# Autodesk Inventor assembly: złożenie czołg
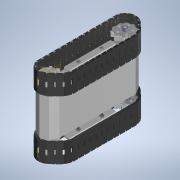
[picture p0: Inventor's stored thumbnail of the model, 180x180]
Saved by Autodesk Inventor 2021 (Build 250183000, 183)
## iProperties
Created: 2021-06-22
Part Number: złożenie czołg
Document SubType Name: Assembly
Designer: Łukasz
Author: Łukasz
## Documents named in this file (10)
- E:\GITHUB_Czołg\Szybki-Czolg-antyRadziecki\złożenie czołg.iam
- E:\GITHUB_Czołg\Szybki-Czolg-antyRadziecki\złożenie gąsienicy lewej.iam
- E:\GITHUB_Czołg\Szybki-Czolg-antyRadziecki\złożenie gąsienicy prawej.iam
- C:\Users\Łukasz\Documents\Inventor\Content Center Files\R2021\en-US\AS 1237 (3.1)\AS 1237 - 12 mm(1)Aluminium-6061.ipt
- C:\Users\Łukasz\Documents\Inventor\Content Center Files\R2021\en-US\BS 292 (I)\BS 292 Part 1 - 6001 - 12 x 28 x 8.ipt
- E:\GITHUB_Czołg\Szybki-Czolg-antyRadziecki\rama.ipt
- E:\GITHUB_Czołg\Szybki-Czolg-antyRadziecki\dystans na łożysk 6001 19mm.ipt
- E:\GITHUB_Czołg\Szybki-Czolg-antyRadziecki\blokada osi.ipt
- C:\Users\Łukasz\Documents\Inventor\Content Center Files\R2021\en-US\KS B 1002  C (2)\KS B 1002 - C  M 8 x 60(1).ipt
- C:\Users\Łukasz\Documents\Inventor\Content Center Files\R2021\en-US\AS 1474(1)\AS 1474 - M8(1).ipt
## Components (31 placed, 9 different names)
1. złożenie gąsienicy lewej:1 [sub-assembly] — Flush:2, Flush:3, Mate:1, Rotational:1, Rotational:10, Rotational:11, Rotational:17, Rotational:18, Rotational:19, Rotational:20
2. złożenie gąsienicy prawej:1 [sub-assembly] — Flush:2, Flush:3, Mate:1, Rigid:1, Angle:1, Rotational:6, Rotational:7, Rotational:21, Rotational:22, Rotational:25, Rotational:26
3. AS 1237 (3.1) 12 mm - Aluminum 6061:1 — Rigid:1, Rotational:5
4. AS 1237 (3.1) 12 mm - Aluminum 6061:2 — Rotational:1
5. BS 292: Part 1 (I) (Metric) 6001 - 12 x 28 x 8:1 — Rotational:2, Rotational:3, Rotational:5
6. BS 292: Part 1 (I) (Metric) 6001 - 12 x 28 x 8:2 — Rotational:4
7. rama:1 — Rotational:2, Angle:1, Rigid:2, Rigid:3, Rotational:12, Rotational:13, Rotational:14, Rotational:15, Rotational:16, Rotational:23, Rotational:24
8. dystans na łożysk 6001 19mm:1 — Rotational:3, Rotational:4
9. blokada osi:1 — Rotational:6
10. blokada osi:2 — Rotational:7
11. dystans na łożysk 6001 19mm:2 — Rotational:8, Rotational:9
12. BS 292: Part 1 (I) (Metric) 6001 - 12 x 28 x 8:3 — Rotational:9
13. BS 292: Part 1 (I) (Metric) 6001 - 12 x 28 x 8:4 — Rigid:2, Rotational:8
14. blokada osi:3 — Rotational:11
15. blokada osi:4 — Rotational:10
16. KS B 1002 C Regular Thread (Full Threaded) C  M 8 x 60:1 — Rotational:12
17. KS B 1002 C Regular Thread (Full Threaded) C  M 8 x 60:2 — Rotational:14
18. KS B 1002 C Regular Thread (Full Threaded) C  M 8 x 60:3 — Rigid:3
19. KS B 1002 C Regular Thread (Full Threaded) C  M 8 x 60:4 — Rotational:13
20. AS 1474 - Metric M8:1 — Rotational:20
21. AS 1474 - Metric M8:2 — Rotational:21
22. AS 1474 - Metric M8:3 — Rotational:23
23. AS 1474 - Metric M8:4 — Rotational:22
24. AS 1474 - Metric M8:5 — Rotational:26
25. AS 1474 - Metric M8:6 — Rotational:24
26. AS 1474 - Metric M8:7 — Rotational:19
27. AS 1474 - Metric M8:8 — Rotational:25
28. AS 1474 - Metric M8:9 — Rotational:17
29. AS 1474 - Metric M8:10 — Rotational:18
30. AS 1474 - Metric M8:11 — Rotational:15
31. AS 1474 - Metric M8:12 — Rotational:16
## Relationships (33: RevoluteJoint 26, WeldJoint 3, Flush 2, Mate 1, Angle 1)
- Flush:2: złożenie gąsienicy lewej:1 ↔ złożenie gąsienicy prawej:1
- Flush:3: złożenie gąsienicy lewej:1 ↔ złożenie gąsienicy prawej:1
- Mate:1 (170 mm): złożenie gąsienicy lewej:1 ↔ złożenie gąsienicy prawej:1
- Rigid:1 [WeldJoint]: złożenie gąsienicy prawej:1 ↔ AS 1237 (3.1) 12 mm - Aluminum 6061:1
- Rotational:1 [RevoluteJoint]: złożenie gąsienicy lewej:1 ↔ AS 1237 (3.1) 12 mm - Aluminum 6061:2
- Rotational:2 [RevoluteJoint]: BS 292: Part 1 (I) (Metric) 6001 - 12 x 28 x 8:1 ↔ rama:1
- Rotational:3 [RevoluteJoint]: BS 292: Part 1 (I) (Metric) 6001 - 12 x 28 x 8:1 ↔ dystans na łożysk 6001 19mm:1
- Rotational:4 [RevoluteJoint]: BS 292: Part 1 (I) (Metric) 6001 - 12 x 28 x 8:2 ↔ dystans na łożysk 6001 19mm:1
- Rotational:5 [RevoluteJoint]: AS 1237 (3.1) 12 mm - Aluminum 6061:1 ↔ BS 292: Part 1 (I) (Metric) 6001 - 12 x 28 x 8:1
- Angle:1 (0 deg): złożenie gąsienicy prawej:1 ↔ rama:1
- Rotational:6 [RevoluteJoint]: złożenie gąsienicy prawej:1 ↔ blokada osi:1
- Rotational:7 [RevoluteJoint]: złożenie gąsienicy prawej:1 ↔ blokada osi:2
- Rigid:2 [WeldJoint]: rama:1 ↔ BS 292: Part 1 (I) (Metric) 6001 - 12 x 28 x 8:4
- Rotational:8 [RevoluteJoint]: dystans na łożysk 6001 19mm:2 ↔ BS 292: Part 1 (I) (Metric) 6001 - 12 x 28 x 8:4
- Rotational:9 [RevoluteJoint]: dystans na łożysk 6001 19mm:2 ↔ BS 292: Part 1 (I) (Metric) 6001 - 12 x 28 x 8:3
- Rotational:10 [RevoluteJoint]: złożenie gąsienicy lewej:1 ↔ blokada osi:4
- Rotational:11 [RevoluteJoint]: złożenie gąsienicy lewej:1 ↔ blokada osi:3
- Rigid:3 [WeldJoint]: rama:1 ↔ KS B 1002 C Regular Thread (Full Threaded) C  M 8 x 60:3
- Rotational:12 [RevoluteJoint]: rama:1 ↔ KS B 1002 C Regular Thread (Full Threaded) C  M 8 x 60:1
- Rotational:13 [RevoluteJoint]: rama:1 ↔ KS B 1002 C Regular Thread (Full Threaded) C  M 8 x 60:4
- Rotational:14 [RevoluteJoint]: rama:1 ↔ KS B 1002 C Regular Thread (Full Threaded) C  M 8 x 60:2
- Rotational:15 [RevoluteJoint]: rama:1 ↔ AS 1474 - Metric M8:11
- Rotational:16 [RevoluteJoint]: rama:1 ↔ AS 1474 - Metric M8:12
- Rotational:17 [RevoluteJoint]: złożenie gąsienicy lewej:1 ↔ AS 1474 - Metric M8:9
- Rotational:18 [RevoluteJoint]: złożenie gąsienicy lewej:1 ↔ AS 1474 - Metric M8:10
- Rotational:19 [RevoluteJoint]: złożenie gąsienicy lewej:1 ↔ AS 1474 - Metric M8:7
- Rotational:20 [RevoluteJoint]: złożenie gąsienicy lewej:1 ↔ AS 1474 - Metric M8:1
- Rotational:21 [RevoluteJoint]: złożenie gąsienicy prawej:1 ↔ AS 1474 - Metric M8:2
- Rotational:22 [RevoluteJoint]: złożenie gąsienicy prawej:1 ↔ AS 1474 - Metric M8:4
- Rotational:23 [RevoluteJoint]: rama:1 ↔ AS 1474 - Metric M8:3
- Rotational:24 [RevoluteJoint]: rama:1 ↔ AS 1474 - Metric M8:6
- Rotational:25 [RevoluteJoint]: złożenie gąsienicy prawej:1 ↔ AS 1474 - Metric M8:8
- Rotational:26 [RevoluteJoint]: złożenie gąsienicy prawej:1 ↔ AS 1474 - Metric M8:5
